# Autodesk Inventor assembly: SCCJ10-5
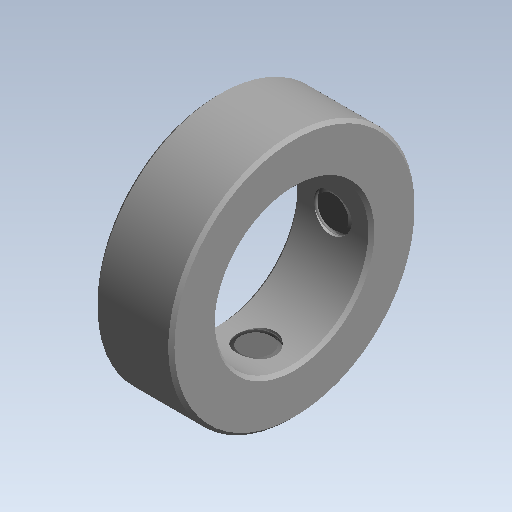
[picture p0: Inventor's stored thumbnail of the model, 512x512]
Saved by Autodesk Inventor 2020 (Build 240168000, 168)
## iProperties
Part Number: SCCJ10-5
Catalog Web Link: www.cadenas.de
Description: SCCJ, PSCCJ, SSCCJ-Set Collars - Set Screw - Standard Compact Type/2-Hole Type
Vendor: MISUMI
Document SubType Name: Assembly
Designer: partserver
Manufacturer: MISUMI
Mass: 0.613913 g
Surface Area: 7.47007 cm^2
Volume: 0.613913 cm^3
Density: 1 g/cm^3
Category: PARTsolutions
Company: MISUMI
PSOL_IDENT_0: {$CADENAS_DATA\23d-libs\misumi\metric\03_set_collars\sccj_asmtab.prj},193 {VTYP=3D},{STYP=ASSTAB},{N
PSOL_IDENT_1: B=SCCJ10-5},{LINA=SCCJ10-5},{NN=SCCJ, PSCCJ, SSCCJ},{DATE=09.09.2019 15:26:49},{GEOMDATE=28.10.2015
PSOL_IDENT_2: 04:53:08},{VERSION=},{LINEID=40},{WBVAR=MAT,ST,BS},{WBNUMERIC=BS}  {NB=SCCJ10-5},{LINA=SCCJ10-5},{KT=
PSOL_IDENT_3: DUMMY},{PN=SCCJ10-5},{TYPE=SCCJ},{MAT=S45C},{MATALG=  'S45C','1045 Carbon Steel','SUS304','304 Stain
PSOL_IDENT_4: less Steel'    },{ST=B},{STALG=  'B','Black Oxide','ENP','Electroless Nickel Plating'           },{A
PSOL_IDENT_5: C=Set Screw 2 Pcs.},{D=10},{BS=5},{BS1=5},{D1=16},{DD1=0.0},{C=0.2},{SS=M3X3},{M1=3},{M2=3},{PPATH=s
PSOL_IDENT_6: ccj/sccj_templ.prj}
NB: SCCJ10-5
NN: SCCJ, PSCCJ, SSCCJ
NT: Set Collars - Set Screw - Standard Compact Type/2-Hole Type
NBSYN: $PN.
LINA: SCCJ10-5
CATALOG: Misumi
PN: SCCJ10-5
MAT: 1045 Carbon Steel
ST: Black Oxide
AC: Set Screw 2 Pcs.
D: 10
BS: 5
D1: 16
DD1: 0
C: 0.2
SS: M3X3
SUPPLIER: MISUMI
ARTICLENO: SCCJ10-5
BOMINFO: SCCJ10-5
CREATOR: CADENAS GmbH
Title: SCCJ10-5
Author: Cadenas PARTsolutions
Comments: Set Collars - Set Screw - Standard Compact Type/2-Hole Type
## Documents named in this file (3)
- C:\Users\lvglv\Documents\GitHub\Cheap_Belt_Printer\Model\Parts\MISUMI\SCCJ10-5_Autodesk_Inventor_2020_20201011\AIS2020\SCCJ10-5.iam
- C:\Users\lvglv\Documents\GitHub\Cheap_Belt_Printer\Model\Parts\MISUMI\SCCJ10-5_Autodesk_Inventor_2020_20201011\AIS2020\SCCJ10-5_b.ipt
- C:\Users\lvglv\Documents\GitHub\Cheap_Belt_Printer\Model\Parts\MISUMI\SCCJ10-5_Autodesk_Inventor_2020_20201011\AIS2020\Hexagon socket set screw with flat point DIN 913 - M3x3.ipt
## Components (3 placed, 2 different names)
1. SCCJ10-5_b:1 — to_screw1_Z@1 <-> IP2_Z@2, to_screw1_YZ@1 <-> IP2_YZ@2, to_screw2_Z@1 <-> IP2_Z@3, to_screw2_YZ@1 <-> IP2_YZ@3
2. Hexagon socket set screw with flat point DIN 913 - M3x3:1 — to_screw1_Z@1 <-> IP2_Z@2, to_screw1_YZ@1 <-> IP2_YZ@2
3. Hexagon socket set screw with flat point DIN 913 - M3x3:2 — to_screw2_Z@1 <-> IP2_Z@3, to_screw2_YZ@1 <-> IP2_YZ@3
## Relationships (4: Mate 2, Angle 2)
- to_screw1_Z@1 <-> IP2_Z@2 [Mate]: SCCJ10-5_b:1 ↔ Hexagon socket set screw with flat point DIN 913 - M3x3:1
- to_screw1_YZ@1 <-> IP2_YZ@2 [Angle] (0 deg): SCCJ10-5_b:1 ↔ Hexagon socket set screw with flat point DIN 913 - M3x3:1
- to_screw2_Z@1 <-> IP2_Z@3 [Mate]: SCCJ10-5_b:1 ↔ Hexagon socket set screw with flat point DIN 913 - M3x3:2
- to_screw2_YZ@1 <-> IP2_YZ@3 [Angle] (0 deg): SCCJ10-5_b:1 ↔ Hexagon socket set screw with flat point DIN 913 - M3x3:2
